# Autodesk Inventor assembly: HS 60T Gear, Circle_MIR
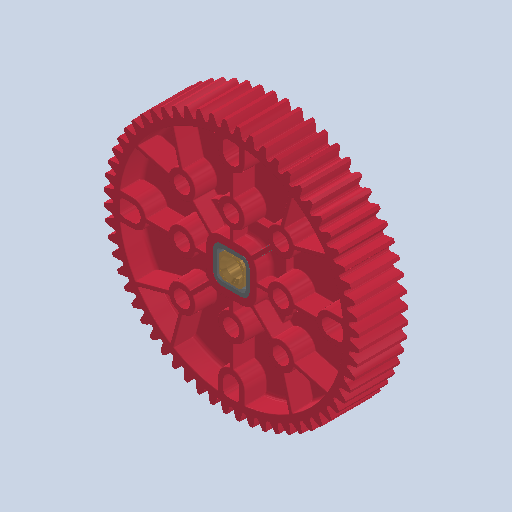
[picture p0: Inventor's stored thumbnail of the model, 512x512]
Saved by Autodesk Inventor 2024 (Build 280153000, 153)
## iProperties
Created: 2022-08-02
Part Number: HS 60T Gear, Circle_MIR
Document SubType Name: Assembly
Designer: ismae
Author: ylu12
## Documents named in this file (3)
- C:\Users\ismae\Desktop\VEX\CAD 2023\VEX-CAD-Inventor\Motion\Gears\HS Gear\HS 60T Gear, Circle_MIR.iam
- C:\Users\ismae\Desktop\VEX\CAD 2023\VEX-CAD-Inventor\Motion\HS Shaft Adapter Circle_MIR3.ipt
- C:\Users\ismae\Desktop\VEX\CAD 2023\VEX-CAD-Inventor\Motion\Gears\Reference Files\HS 60T Gear, No Insert_MIR.ipt
## Components (2 placed, 2 different names)
1. HS Shaft Adapter Circle_MIR3:1 — Nivelación:1, Coincidencia:2, Coincidencia:1
2. HS 60T Gear, No Insert_MIR:1 — Coincidencia:14, Coincidencia:13, Nivelación:7
## Relationships (6: Mate 4, Flush 2)
- Nivelación:1 [Flush] (-6.35 mm): HS Shaft Adapter Circle_MIR3:1
- Coincidencia:2 [Mate]: HS Shaft Adapter Circle_MIR3:1
- Coincidencia:1 [Mate]: HS Shaft Adapter Circle_MIR3:1
- Coincidencia:14 [Mate]: HS 60T Gear, No Insert_MIR:1
- Coincidencia:13 [Mate]: HS 60T Gear, No Insert_MIR:1
- Nivelación:7 [Flush]: HS 60T Gear, No Insert_MIR:1
